# Autodesk Inventor assembly: DoublePulley
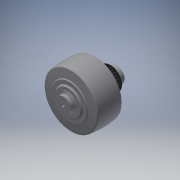
[picture p0: Inventor's stored thumbnail of the model, 180x180]
Saved by Autodesk Inventor 2016 (Build 200138000, 138)
## iProperties
Created: 2017-01-15
Part Number: DoublePulley
Document SubType Name: Assembly
Designer: Kyle
Author: Kyle
## Documents named in this file (7)
- F:\FRC\2017\DriveTrainRev2\Individual Parts\DoublePulley.iam
- F:\FRC\2017\DriveTrainRev2\Individual Parts\.5Bearing.ipt
- F:\FRC\2017\DriveTrainRev2\Individual Parts\3.875Churro.ipt
- F:\FRC\2017\DriveTrainRev2\Individual Parts\4x2Colson.ipt
- F:\FRC\2017\DriveTrainRev2\Individual Parts\24t9MMPulley6mm.ipt
- F:\FRC\2017\DriveTrainRev2\Individual Parts\24t9MMPulleyExtension.ipt
- F:\FRC\2017\DriveTrainRev2\Individual Parts\.106Spacer.ipt
## Components (8 placed, 6 different names)
1. .5Bearing:1 — Mate:1, Flush:1, Mate:3
2. 3.875Churro:1 — Mate:1, Flush:1, Mate:2, Mate:10, Mate:12, Mate:14
3. 4x2Colson:1 — Mate:2, Mate:3, Mate:11
4. 24t9MMPulley6mm:1 — Mate:4, Mate:5, Mate:6, Mate:7, Mate:11
5. 24t9MMPulley6mm:2 — Mate:7, Mate:8, Mate:9, Mate:10, Mate:13
6. 24t9MMPulleyExtension:1 — Mate:4, Mate:5, Mate:6, Mate:8, Mate:9
7. .106Spacer:1 — Mate:12, Mate:13, Mate:15
8. .5Bearing:2 — Mate:14, Mate:15
## Relationships (16: Mate 15, Flush 1)
- Mate:1: .5Bearing:1 ↔ 3.875Churro:1
- Flush:1: .5Bearing:1 ↔ 3.875Churro:1
- Mate:2: 3.875Churro:1 ↔ 4x2Colson:1
- Mate:3: .5Bearing:1 ↔ 4x2Colson:1
- Mate:4: 24t9MMPulley6mm:1 ↔ 24t9MMPulleyExtension:1
- Mate:5: 24t9MMPulley6mm:1 ↔ 24t9MMPulleyExtension:1
- Mate:6: 24t9MMPulley6mm:1 ↔ 24t9MMPulleyExtension:1
- Mate:7: 24t9MMPulley6mm:1 ↔ 24t9MMPulley6mm:2
- Mate:8: 24t9MMPulley6mm:2 ↔ 24t9MMPulleyExtension:1
- Mate:9: 24t9MMPulley6mm:2 ↔ 24t9MMPulleyExtension:1
- Mate:10: 3.875Churro:1 ↔ 24t9MMPulley6mm:2
- Mate:11: 4x2Colson:1 ↔ 24t9MMPulley6mm:1
- Mate:12: 3.875Churro:1 ↔ .106Spacer:1
- Mate:13: 24t9MMPulley6mm:2 ↔ .106Spacer:1
- Mate:14: 3.875Churro:1 ↔ .5Bearing:2
- Mate:15: .106Spacer:1 ↔ .5Bearing:2
